# Autodesk Inventor assembly: MG-Ballsensor
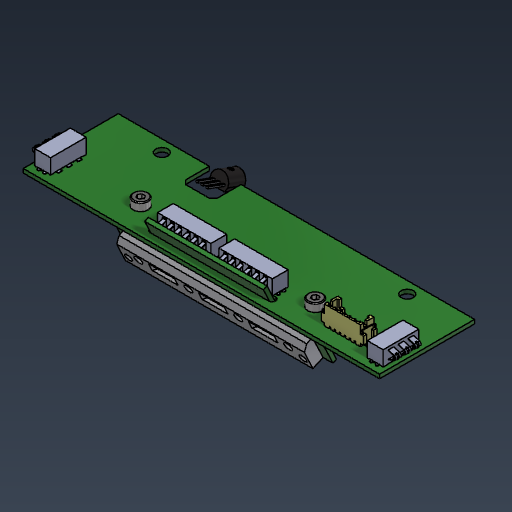
[picture p0: Inventor's stored thumbnail of the model, 512x512]
Saved by Autodesk Inventor 2023.1 (Build 271208000, 208)
## iProperties
Part Number: MG-Ballsensor
Material: Generisch
Document SubType Name: Assembly
Designer: rYan
Mass: 6.53598 g
Surface Area: 102.826 cm^2
Volume: 4.91918 cm^3
Density: 1.32867 g/cm^3
Author: rYan
## Documents named in this file (8)
- D:\TIGERsGIT\Hardware\mechanik\2024\Inventor\Robot\Electronics\MG-Ballsensor.iam
- D:\TIGERsGIT\Hardware\mechanik\2024\Inventor\Purchased Parts\AVX Interconnect 00-9155-003-541-006.ipt
- D:\TIGERsGIT\Hardware\mechanik\2024\Inventor\Purchased Parts\DF13C-6P-1.25V.ipt
- D:\TIGERsGIT\Hardware\mechanik\2024\Inventor\Robot\Electronics\Ballsensorplatine.ipt
- D:\TIGERsGIT\Hardware\mechanik\2024\Inventor\Robot\Electronics\MG-Ballsensorplatine.iam
- D:\TIGERsGIT\Hardware\mechanik\2024\Inventor\Inhaltscenter\de-DE\ISO 4762(2)\ISO 4762 - M2 x 4ISO.ipt
- D:\TIGERsGIT\Hardware\mechanik\2024\Inventor\Purchased Parts\AVX Interconnect 00-9155-006-741-006.ipt
- D:\TIGERsGIT\Hardware\mechanik\2024\Inventor\Purchased Parts\TO-92.ipt
## Components (10 placed, 7 different names)
1. Ballsensorplatine:1 — Fluchtend:1, Fluchtend:2, Fluchtend:3, Fluchtend:4, Fluchtend:5, Passend:1, Passend:2, Fluchtend:7, Passend:7, Fluchtend:9, Einfügen:2, Passend:8, Einfügen:3, Einfügen:4, Passend:10, Passend:11, Fluchtend:12, Winkel:1
2. AVX Interconnect 00-9155-003-541-006:1 — Fluchtend:4, Passend:2, Fluchtend:8
3. AVX Interconnect 00-9155-003-541-006:2 — Fluchtend:5, Passend:1, Fluchtend:7, Fluchtend:8
4. DF13C-6P-1.25V:1 — Passend:7, Fluchtend:9
5. MG-Ballsensorplatine:1 [sub-assembly] — Einfügen:2, Passend:8
6. ISO 4762 M2 x 4:1 — Einfügen:3
7. ISO 4762 M2 x 4:3 — Einfügen:4
8. AVX Interconnect 00-9155-006-741-006:1 — Passend:10, Passend:12, Fluchtend:11
9. AVX Interconnect 00-9155-006-741-006:2 — Passend:11, Fluchtend:10, Fluchtend:11, Fluchtend:12
10. TO-92:1 — Winkel:1, Fluchtend:14
## Relationships (23: Flush 12, Mate 7, Insert 3, Angle 1)
- Fluchtend:1 [Flush]: Ballsensorplatine:1
- Fluchtend:2 [Flush]: Ballsensorplatine:1
- Fluchtend:3 [Flush]: Ballsensorplatine:1
- Fluchtend:4 [Flush] (1 mm): Ballsensorplatine:1 ↔ AVX Interconnect 00-9155-003-541-006:1
- Fluchtend:5 [Flush] (1 mm): Ballsensorplatine:1 ↔ AVX Interconnect 00-9155-003-541-006:2
- Passend:1 [Mate]: Ballsensorplatine:1 ↔ AVX Interconnect 00-9155-003-541-006:2
- Passend:2 [Mate]: Ballsensorplatine:1 ↔ AVX Interconnect 00-9155-003-541-006:1
- Fluchtend:7 [Flush] (13.1 mm): Ballsensorplatine:1 ↔ AVX Interconnect 00-9155-003-541-006:2
- Fluchtend:8 [Flush]: AVX Interconnect 00-9155-003-541-006:1 ↔ AVX Interconnect 00-9155-003-541-006:2
- Passend:7 [Mate]: Ballsensorplatine:1 ↔ DF13C-6P-1.25V:1
- Fluchtend:9 [Flush] (-17 mm): Ballsensorplatine:1 ↔ DF13C-6P-1.25V:1
- Einfügen:2 [Insert]: Ballsensorplatine:1 ↔ MG-Ballsensorplatine:1
- Passend:8 [Mate]: Ballsensorplatine:1 ↔ MG-Ballsensorplatine:1
- Einfügen:3 [Insert]: Ballsensorplatine:1 ↔ ISO 4762 M2 x 4:1
- Einfügen:4 [Insert]: Ballsensorplatine:1 ↔ ISO 4762 M2 x 4:3
- Passend:10 [Mate]: Ballsensorplatine:1 ↔ AVX Interconnect 00-9155-006-741-006:1
- Passend:11 [Mate]: Ballsensorplatine:1 ↔ AVX Interconnect 00-9155-006-741-006:2
- Fluchtend:10 [Flush] (-1 mm): AVX Interconnect 00-9155-006-741-006:2
- Passend:12 [Mate] (1 mm): AVX Interconnect 00-9155-006-741-006:1
- Fluchtend:11 [Flush]: AVX Interconnect 00-9155-006-741-006:1 ↔ AVX Interconnect 00-9155-006-741-006:2
- Fluchtend:12 [Flush] (0.4 mm): Ballsensorplatine:1 ↔ AVX Interconnect 00-9155-006-741-006:2
- Winkel:1 [Angle] (110 deg): Ballsensorplatine:1 ↔ TO-92:1
- Fluchtend:14 [Flush] (-18 mm): TO-92:1
